# Autodesk Inventor assembly: caster
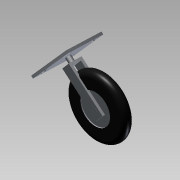
[picture p0: Inventor's stored thumbnail of the model, 180x180]
Saved by Autodesk Inventor 2012 (Build 160160000, 160)
## iProperties
Created: 2012-09-15
Part Number: caster
Document SubType Name: Assembly
Designer: Admin
Author: Admin
## Documents named in this file (4)
- C:\Users\Admin\Documents\Inventor\Robotics 2013\Cart\pneumatic caster\caster.iam
- C:\Users\Admin\Documents\Inventor\Robotics 2013\Cart\pneumatic caster\wheel.ipt
- C:\Users\Admin\Documents\Inventor\Robotics 2013\Cart\pneumatic caster\wheel support.ipt
- C:\Users\Admin\Documents\Inventor\Robotics 2013\Cart\pneumatic caster\wheel mount plate.ipt
## Components (3 placed, 3 different names)
1. wheel:1 — Mate:1, Mate:2
2. wheel support:1 — Mate:1, Mate:2, Mate:3, Flush:1
3. wheel mount plate:1 — Mate:3, Flush:1
## Relationships (4: Mate 3, Flush 1)
- Mate:1: wheel:1 ↔ wheel support:1
- Mate:2: wheel:1 ↔ wheel support:1
- Mate:3: wheel support:1 ↔ wheel mount plate:1
- Flush:1: wheel support:1 ↔ wheel mount plate:1
